# Autodesk Inventor assembly: финальная сборка
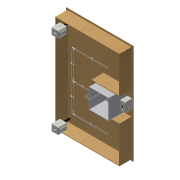
[picture p0: Inventor's stored thumbnail of the model, 180x180]
Saved by Autodesk Inventor 2021 (Build 250183000, 183)
## iProperties
Created: 2023-02-17
Part Number: финальная сборка
Document SubType Name: Assembly
Designer: Tasya
Author: Tasya
## Documents named in this file (10)
- C:\Users\Tasya\Desktop\теплица\3D\Сборки iam\финальная сборка.iam
- C:\Users\Tasya\Desktop\теплица\датчики почва воздух\компановка новая.iam
- C:\Users\Tasya\Desktop\теплица\основание\сборка основание.iam
- C:\Users\Tasya\Desktop\теплица\grabcad\Water Level Sensor.ipt
- C:\Users\Tasya\Desktop\теплица\емкость\УвлажнительНовый.ipt
- C:\Users\Tasya\Desktop\теплица\емкость\насос.ipt
- C:\Users\Tasya\Desktop\теплица\емкость\держатель.ipt
- C:\Users\Tasya\Desktop\теплица\основание\стенка 2.ipt
- C:\Users\Tasya\Desktop\теплица\основание\стенка 3.ipt
- C:\Users\Tasya\Desktop\теплица\основание\стенка боковая.ipt
## Components (14 placed, 9 different names)
1. компановка новая:1 [sub-assembly] — Совмещение:1, Совмещение:2, Совмещение:3, Заподлицо:3, Заподлицо:4
2. сборка основание:1 [sub-assembly] — Совмещение:1, Совмещение:2, Совмещение:3, Совмещение:6, Совмещение:7, Совмещение:8, Угол:1, Угол:2, Совмещение:9, Угол:3, Совмещение:10, Совмещение:11, Заподлицо:2, Совмещение:12, Совмещение:13, Угол:4, Совмещение:14, Угол:5, Совмещение:15, Совмещение:16, Совмещение:17, Угол:6, Совмещение:18, Совмещение:19, Заподлицо:5, Совмещение:20, Совмещение:22, Совмещение:23, Совмещение:24, Совмещение:25
3. Water Level Sensor:1
4. УвлажнительНовый:1
5. насос:1 — Совмещение:6, Совмещение:7, Совмещение:8, Угол:1
6. держатель:1 — Угол:2, Совмещение:9, Заподлицо:2
7. держатель:2 — Угол:3, Совмещение:10, Совмещение:11
8. держатель:3 — Совмещение:14, Угол:5, Совмещение:15
9. держатель:4 — Совмещение:12, Совмещение:13, Угол:4
10. держатель:5 — Совмещение:16, Совмещение:17, Угол:6
11. компановка новая:2 [sub-assembly] — Заподлицо:3, Заподлицо:4, Совмещение:26
12. стенка 2:1 — Совмещение:20, Совмещение:21, Совмещение:22
13. стенка 3:1 — Совмещение:23, Совмещение:24, Совмещение:25
14. стенка боковая:1 — Совмещение:18, Совмещение:19, Заподлицо:5, Совмещение:21, Совмещение:26
## Relationships (34: Mate 24, Angle 6, Flush 4)
- Совмещение:1 [Mate] (75 mm): компановка новая:1 ↔ сборка основание:1
- Совмещение:2 [Mate] (20 mm): компановка новая:1 ↔ сборка основание:1
- Совмещение:3 [Mate] (20 mm): компановка новая:1 ↔ сборка основание:1
- Совмещение:6 [Mate]: сборка основание:1 ↔ насос:1
- Совмещение:7 [Mate] (10 mm): сборка основание:1 ↔ насос:1
- Совмещение:8 [Mate] (45 mm): сборка основание:1 ↔ насос:1
- Угол:1 [Angle] (0 deg): сборка основание:1 ↔ насос:1
- Угол:2 [Angle] (180 deg): сборка основание:1 ↔ держатель:1
- Совмещение:9 [Mate]: сборка основание:1 ↔ держатель:1
- Угол:3 [Angle] (180 deg): сборка основание:1 ↔ держатель:2
- Совмещение:10 [Mate]: сборка основание:1 ↔ держатель:2
- Совмещение:11 [Mate] (81.5 mm): сборка основание:1 ↔ держатель:2
- Заподлицо:2 [Flush] (116 mm): сборка основание:1 ↔ держатель:1
- Совмещение:12 [Mate]: сборка основание:1 ↔ держатель:4
- Совмещение:13 [Mate] (81.5 mm): сборка основание:1 ↔ держатель:4
- Угол:4 [Angle] (180 deg): сборка основание:1 ↔ держатель:4
- Совмещение:14 [Mate]: сборка основание:1 ↔ держатель:3
- Угол:5 [Angle] (0 deg): сборка основание:1 ↔ держатель:3
- Совмещение:15 [Mate] (50 mm): сборка основание:1 ↔ держатель:3
- Совмещение:16 [Mate]: сборка основание:1 ↔ держатель:5
- Совмещение:17 [Mate] (116 mm): сборка основание:1 ↔ держатель:5
- Угол:6 [Angle] (0 deg): сборка основание:1 ↔ держатель:5
- Заподлицо:3 [Flush]: компановка новая:1 ↔ компановка новая:2
- Заподлицо:4 [Flush]: компановка новая:1 ↔ компановка новая:2
- Совмещение:18 [Mate]: сборка основание:1 ↔ стенка боковая:1
- Совмещение:19 [Mate]: сборка основание:1 ↔ стенка боковая:1
- Заподлицо:5 [Flush]: сборка основание:1 ↔ стенка боковая:1
- Совмещение:20 [Mate]: сборка основание:1 ↔ стенка 2:1
- Совмещение:21 [Mate]: стенка 2:1 ↔ стенка боковая:1
- Совмещение:22 [Mate]: сборка основание:1 ↔ стенка 2:1
- Совмещение:23 [Mate]: сборка основание:1 ↔ стенка 3:1
- Совмещение:24 [Mate]: сборка основание:1 ↔ стенка 3:1
- Совмещение:25 [Mate]: сборка основание:1 ↔ стенка 3:1
- Совмещение:26 [Mate] (20 mm): компановка новая:2 ↔ стенка боковая:1
